# Autodesk Inventor assembly: drivebase V2
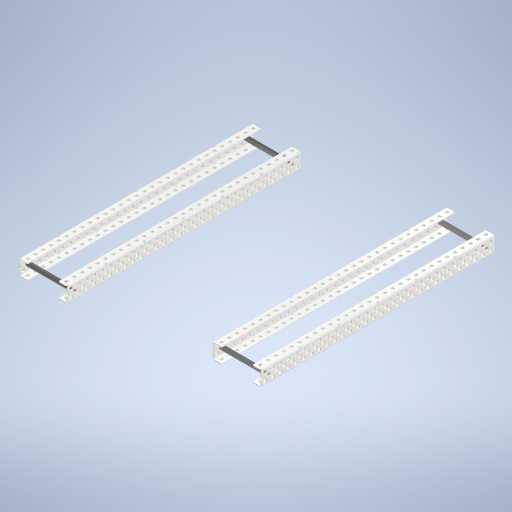
[picture p0: Inventor's stored thumbnail of the model, 512x512]
Saved by Autodesk Inventor 2023 (Build 270158000, 158)
## iProperties
Created: 2023-11-07
Part Number: drivebase V2
Document SubType Name: Assembly
Designer: Robodox
Author: Robodox
## Documents named in this file (4)
- C:\Users\Robodox\Documents\GitHub\2023-599Z\BBotCAD\drivebase V2.iam
- C:\Users\Robodox\Documents\GitHub\2023-599Z\BBotCAD\VEX-CAD-Inventor-1.4.0\Structure\C Channel\Aluminum 1x2x1\Alu C 1x2x1x30.ipt
- C:\Users\Robodox\Documents\GitHub\2023-599Z\BBotCAD\VEX-CAD-Inventor-1.4.0\Structure\Standoff.ipt
- C:\Users\Robodox\Documents\GitHub\2023-599Z\BBotCAD\VEX-CAD-Inventor-1.4.0\Structure\Standoff\Standoff 3.00.ipt
## Components (8 placed, 2 different names)
1. Alu C 1x2x1x30:1 — Mate:4, Mate:5
2. Alu C 1x2x1x30:2 — Mate:2, Mate:6
3. Alu C 1x2x1x30:3 — Mate:3
4. Alu C 1x2x1x30:4 — Mate:1
5. Standoff 3.00:1 — Mate:3, Mate:4
6. Standoff 3.00:2 — Mate:1, Mate:2
7. Standoff 3.00:3 — Mate:5
8. Standoff 3.00:4 — Mate:6
## Relationships (6: Mate 6)
- Mate:1: Alu C 1x2x1x30:4 ↔ Standoff 3.00:2
- Mate:2: Alu C 1x2x1x30:2 ↔ Standoff 3.00:2
- Mate:3: Alu C 1x2x1x30:3 ↔ Standoff 3.00:1
- Mate:4: Alu C 1x2x1x30:1 ↔ Standoff 3.00:1
- Mate:5: Alu C 1x2x1x30:1 ↔ Standoff 3.00:3
- Mate:6: Alu C 1x2x1x30:2 ↔ Standoff 3.00:4
